# Autodesk Inventor assembly: Pancake_Top Board Assy
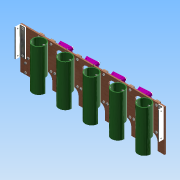
[picture p0: Inventor's stored thumbnail of the model, 180x180]
Saved by Autodesk Inventor 2018.1 (Build 221171000, 171)
## iProperties
Created: 2019-02-21
Part Number: Pancake_Top Board Assy
Document SubType Name: Assembly
Designer: James
Author: James
## Documents named in this file (18)
- C:\Users\admin\Desktop\Ball-Machine\Pancake Sort\Pancake_Top Board Assy.iam
- C:\Users\admin\Desktop\Ball-Machine\Pancake Sort\Pancake_Top Board.ipt
- C:\Users\admin\Desktop\Ball-Machine\Pancake Sort\Pancake_Angle Bracket 2.ipt
- C:\Users\admin\Desktop\Ball-Machine\Pancake Sort\Nyloc Nut - M4.ipt
- C:\Users\admin\Desktop\Ball-Machine\Pancake Sort\Socket Csk Screw - (A2) - M4 x  12.ipt
- C:\Users\admin\Desktop\Ball-Machine\Pancake Sort\Pancake_Side Piece.ipt
- C:\Users\admin\Desktop\Ball-Machine\Pancake Sort\Socket Csk Screw - (A2) - M4 x  16.ipt
- C:\Users\admin\Desktop\Ball-Machine\Pancake Sort\Pancake_Side Piece Short.ipt
- C:\Users\admin\Desktop\Ball-Machine\Pancake Sort\Pancake_Lower Pipe.ipt
- C:\Users\admin\Desktop\Ball-Machine\Pancake Sort\Pancake_Side Piece Short 2.ipt
- C:\Users\admin\Desktop\Ball-Machine\Pancake Sort\Socket Csk Screw - (A2) - M4 x  20.ipt
- C:\Users\admin\Desktop\Ball-Machine\Pancake Sort\Pancake_Side Piece Short 3.ipt
- C:\Users\admin\Desktop\Ball-Machine\Pancake Sort\Pancake_Switch Lever.ipt
- C:\Users\admin\Desktop\Ball-Machine\Pancake Sort\Pancake_Lever Mount Piece.ipt
- C:\Users\admin\Desktop\Ball-Machine\Selection Sort\Selection_Washer.ipt
- C:\Users\admin\Desktop\Ball-Machine\Pancake Sort\Socket Csk Screw - (A2) - M3 x  10.ipt
- C:\Users\admin\Desktop\Ball-Machine\Pancake Sort\Socket Cap Screw - Standard - (A2) - M3 x 8.ipt
- C:\Users\admin\Desktop\Ball-Machine\Pancake Sort\Pancake_Eye Screw.ipt
## Components (126 placed, 17 different names)
1. Pancake_Top Board:1 — Flush:1, Flush:2, Flush:3, Mate:1, Mate:2, Mate:3, Flush:4, Mate:4, Mate:5, Mate:6, Flush:5, Mate:7, Mate:8, Tangent:1, Tangent:2, Mate:13, Mate:14, Tangent:3, Tangent:4, Mate:19, Mate:20, Mate:21, Flush:6, Mate:24, Mate:25, Mate:28, Mate:29, Mate:30, Mate:35, Mate:36, Tangent:9, Mate:37, Mate:38, Angle:1, Mate:41, Mate:42, Tangent:10, Tangent:11, Mate:43, Mate:44, Mate:45, Mate:46, Mate:47, Mate:48, Mate:49, Mate:50, Mate:53, Mate:54, Mate:55, Mate:60, Mate:61, Mate:63, Mate:76, Mate:77, Mate:81, Tangent:19, Mate:84, Mate:85, Mate:86, Mate:87
2. Pancake_Angle Bracket 2:1 — Mate:1, Mate:2, Mate:3, Flush:4, Mate:9, Mate:10
3. Pancake_Angle Bracket 2:2 — Mate:4, Mate:5, Mate:6, Flush:5, Mate:15, Mate:16
4. Pancake_Side Piece Short 2:1 — Mate:44, Mate:45, Mate:46, Tangent:12, Tangent:13
5. Nyloc Nut - M4:35 — Mate:49, Mate:52
6. Socket Csk Screw - (A2) - M4 x  16:11 — Mate:47, Tangent:12, Mate:51
7. Nyloc Nut - M4:36 — Mate:50, Mate:51
8. Socket Csk Screw - (A2) - M4 x  16:12 — Mate:48, Tangent:13, Mate:52
9. Pancake_Side Piece Short 3:1 — Mate:53, Mate:54, Mate:55, Mate:58, Mate:59, Tangent:14, Tangent:15
10. Socket Csk Screw - (A2) - M4 x  16:13 — Mate:58, Tangent:14
11. Nyloc Nut - M4:37 — Mate:61
12. Socket Csk Screw - (A2) - M4 x  16:14 — Mate:59, Tangent:15
13. Nyloc Nut - M4:38 — Mate:60
14. Nyloc Nut - M4:1 — Mate:9, Mate:12
15. Nyloc Nut - M4:2 — Mate:10, Mate:11
16. Nyloc Nut - M4:3 — Mate:16, Mate:18
17. Nyloc Nut - M4:4 — Mate:15, Mate:17
18. Socket Csk Screw - (A2) - M4 x  12:1 — Mate:7, Tangent:1, Mate:11
19. Socket Csk Screw - (A2) - M4 x  12:2 — Mate:8, Tangent:2, Mate:12
20. Socket Csk Screw - (A2) - M4 x  12:3 — Mate:14, Tangent:3, Mate:17
21. Socket Csk Screw - (A2) - M4 x  12:4 — Mate:13, Tangent:4, Mate:18
22. Socket Csk Screw - (A2) - M4 x  16:2 — Mate:23, Tangent:5, Mate:27
23. Nyloc Nut - M4:6 — Mate:25, Mate:27
24. Socket Csk Screw - (A2) - M4 x  16:1 — Mate:22, Tangent:6, Mate:26
25. Nyloc Nut - M4:5 — Mate:24, Mate:26
26. Pancake_Side Piece:1 — Mate:19, Mate:20, Mate:21, Flush:6, Mate:22, Mate:23, Tangent:5, Tangent:6
27. Socket Csk Screw - (A2) - M4 x  16:3
28. Nyloc Nut - M4:7
29. Socket Csk Screw - (A2) - M4 x  16:4
30. Nyloc Nut - M4:8
31. Pancake_Side Piece:2 — Tangent:16
32. Socket Csk Screw - (A2) - M4 x  16:5
33. Nyloc Nut - M4:9
34. Socket Csk Screw - (A2) - M4 x  16:6
35. Nyloc Nut - M4:10
36. Pancake_Side Piece:3
37. Socket Csk Screw - (A2) - M4 x  16:7
38. Nyloc Nut - M4:11
39. Socket Csk Screw - (A2) - M4 x  16:8
40. Nyloc Nut - M4:12
41. Pancake_Side Piece:4
42. Socket Csk Screw - (A2) - M4 x  16:9
43. Nyloc Nut - M4:13
44. Socket Csk Screw - (A2) - M4 x  16:10
45. Nyloc Nut - M4:14
46. Pancake_Side Piece:5
47. Pancake_Side Piece Short:1 — Mate:28, Mate:29, Mate:30, Mate:33, Mate:34, Tangent:7, Tangent:8
48. Nyloc Nut - M4:15 — Mate:36
49. Socket Csk Screw - (A2) - M4 x  20:1 — Mate:34, Tangent:7
50. Nyloc Nut - M4:16 — Mate:35
51. Socket Csk Screw - (A2) - M4 x  20:6 — Mate:33, Tangent:8
52. Pancake_Side Piece Short:2 — Tangent:18, Mate:88, Mate:89
53. Nyloc Nut - M4:17
54. Socket Csk Screw - (A2) - M4 x  20:2
55. Nyloc Nut - M4:18
56. Socket Csk Screw - (A2) - M4 x  20:7
57. Pancake_Side Piece Short:3
58. Nyloc Nut - M4:19
59. Socket Csk Screw - (A2) - M4 x  20:3
60. Nyloc Nut - M4:20
61. Socket Csk Screw - (A2) - M4 x  20:8
62. Pancake_Side Piece Short:4
63. Nyloc Nut - M4:21
64. Socket Csk Screw - (A2) - M4 x  20:4
65. Nyloc Nut - M4:22
66. Socket Csk Screw - (A2) - M4 x  20:9
67. Pancake_Side Piece Short:5
68. Nyloc Nut - M4:23
69. Socket Csk Screw - (A2) - M4 x  20:5
70. Nyloc Nut - M4:24
71. Socket Csk Screw - (A2) - M4 x  20:10
72. Socket Csk Screw - (A2) - M4 x  12:6 — Mate:42, Tangent:11
73. Nyloc Nut - M4:26 — Mate:43, Flush:8
74. Socket Csk Screw - (A2) - M4 x  12:5 — Mate:41, Tangent:10
75. Nyloc Nut - M4:25 — Flush:8
76. Pancake_Lower Pipe:1 — Tangent:9, Mate:37, Mate:38, Angle:1
77. Socket Csk Screw - (A2) - M4 x  12:7
78. Nyloc Nut - M4:27
79. Socket Csk Screw - (A2) - M4 x  12:8
80. Nyloc Nut - M4:28
81. Pancake_Lower Pipe:2
82. Socket Csk Screw - (A2) - M4 x  12:9
83. Nyloc Nut - M4:29
84. Socket Csk Screw - (A2) - M4 x  12:10
85. Nyloc Nut - M4:30
86. Pancake_Lower Pipe:3
87. Socket Csk Screw - (A2) - M4 x  12:11
88. Nyloc Nut - M4:31
89. Socket Csk Screw - (A2) - M4 x  12:12
90. Nyloc Nut - M4:32
91. Pancake_Lower Pipe:4
92. Socket Csk Screw - (A2) - M4 x  12:13
93. Nyloc Nut - M4:33
94. Socket Csk Screw - (A2) - M4 x  12:14
95. Nyloc Nut - M4:34
96. Pancake_Lower Pipe:5
97. Socket Cap Screw - Standard - (A2) - M3 x 8:1 — Mate:82, Mate:83
98. Selection_Washer:2 — Mate:78, Mate:79, Mate:82, Mate:83
99. Pancake_Switch Lever:1 — Mate:63, Tangent:16, Tangent:18, Mate:80
100. Socket Csk Screw - (A2) - M3 x  10:2 — Mate:81, Tangent:19
101. Pancake_Lever Mount Piece:2 — Mate:76, Mate:77, Mate:78, Mate:79, Mate:80
102. Pancake_Eye Screw:7 — Mate:88, Mate:89
103. Socket Cap Screw - Standard - (A2) - M3 x 8:2
104. Selection_Washer:3
105. Pancake_Switch Lever:2
106. Socket Csk Screw - (A2) - M3 x  10:3
107. Pancake_Lever Mount Piece:3
108. Pancake_Eye Screw:8
109. Socket Cap Screw - Standard - (A2) - M3 x 8:3
110. Selection_Washer:4
111. Pancake_Switch Lever:3
112. Socket Csk Screw - (A2) - M3 x  10:4
113. Pancake_Lever Mount Piece:4
114. Pancake_Eye Screw:9
115. Socket Cap Screw - Standard - (A2) - M3 x 8:4
116. Selection_Washer:5
117. Pancake_Switch Lever:4
118. Socket Csk Screw - (A2) - M3 x  10:5
119. Pancake_Lever Mount Piece:5
120. Pancake_Eye Screw:10
121. Pancake_Eye Screw:1 — Mate:84, Mate:85
122. Pancake_Eye Screw:2 — Mate:86, Mate:87
123. Pancake_Eye Screw:3
124. Pancake_Eye Screw:4
125. Pancake_Eye Screw:5
126. Pancake_Eye Screw:6
## Component patterns: (5 elements, first: Socket Csk Screw - (A2) - M4 x  16:2 + Nyloc Nut - M4:6 + Socket Csk Screw - (A2) - M4 x  16:1 + Nyloc Nut - M4:5 + Pancake_Side Piece:1), (5 elements, first: Pancake_Side Piece Short:1 + Nyloc Nut - M4:15 + Socket Csk Screw - (A2) - M4 x  20:1 + Nyloc Nut - M4:16 + Socket Csk Screw - (A2) - M4 x  20:6), (5 elements, first: Socket Csk Screw - (A2) - M4 x  12:6 + Nyloc Nut - M4:26 + Socket Csk Screw - (A2) - M4 x  12:5 + Nyloc Nut - M4:25 + Pancake_Lower Pipe:1), (4 elements, first: Socket Cap Screw - Standard - (A2) - M3 x 8:1 + Selection_Washer:2 + Pancake_Switch Lever:1 + Socket Csk Screw - (A2) - M3 x  10:2 + Pancake_Lever Mount Piece:2 + Pancake_Eye Screw:7), (3 elements, first: Pancake_Eye Screw:1 + Pancake_Eye Screw:2)
## Relationships (102: Mate 76, Tangent 18, Flush 7, Angle 1)
- Flush:1: Pancake_Top Board:1
- Flush:2: Pancake_Top Board:1
- Flush:3: Pancake_Top Board:1
- Mate:1: Pancake_Top Board:1 ↔ Pancake_Angle Bracket 2:1
- Mate:2: Pancake_Top Board:1 ↔ Pancake_Angle Bracket 2:1
- Mate:3: Pancake_Top Board:1 ↔ Pancake_Angle Bracket 2:1
- Flush:4: Pancake_Top Board:1 ↔ Pancake_Angle Bracket 2:1
- Mate:4: Pancake_Top Board:1 ↔ Pancake_Angle Bracket 2:2
- Mate:5: Pancake_Top Board:1 ↔ Pancake_Angle Bracket 2:2
- Mate:6: Pancake_Top Board:1 ↔ Pancake_Angle Bracket 2:2
- Flush:5: Pancake_Top Board:1 ↔ Pancake_Angle Bracket 2:2
- Mate:7: Pancake_Top Board:1 ↔ Socket Csk Screw - (A2) - M4 x  12:1
- Mate:8: Pancake_Top Board:1 ↔ Socket Csk Screw - (A2) - M4 x  12:2
- Tangent:1: Pancake_Top Board:1 ↔ Socket Csk Screw - (A2) - M4 x  12:1
- Tangent:2: Pancake_Top Board:1 ↔ Socket Csk Screw - (A2) - M4 x  12:2
- Mate:9: Pancake_Angle Bracket 2:1 ↔ Nyloc Nut - M4:1
- Mate:10: Pancake_Angle Bracket 2:1 ↔ Nyloc Nut - M4:2
- Mate:11: Nyloc Nut - M4:2 ↔ Socket Csk Screw - (A2) - M4 x  12:1
- Mate:12: Nyloc Nut - M4:1 ↔ Socket Csk Screw - (A2) - M4 x  12:2
- Mate:13: Pancake_Top Board:1 ↔ Socket Csk Screw - (A2) - M4 x  12:4
- Mate:14: Pancake_Top Board:1 ↔ Socket Csk Screw - (A2) - M4 x  12:3
- Tangent:3: Pancake_Top Board:1 ↔ Socket Csk Screw - (A2) - M4 x  12:3
- Tangent:4: Pancake_Top Board:1 ↔ Socket Csk Screw - (A2) - M4 x  12:4
- Mate:15: Pancake_Angle Bracket 2:2 ↔ Nyloc Nut - M4:4
- Mate:16: Pancake_Angle Bracket 2:2 ↔ Nyloc Nut - M4:3
- Mate:17: Nyloc Nut - M4:4 ↔ Socket Csk Screw - (A2) - M4 x  12:3
- Mate:18: Nyloc Nut - M4:3 ↔ Socket Csk Screw - (A2) - M4 x  12:4
- Mate:19: Pancake_Top Board:1 ↔ Pancake_Side Piece:1
- Mate:20: Pancake_Top Board:1 ↔ Pancake_Side Piece:1
- Mate:21: Pancake_Top Board:1 ↔ Pancake_Side Piece:1
- Flush:6: Pancake_Top Board:1 ↔ Pancake_Side Piece:1
- Mate:22: Socket Csk Screw - (A2) - M4 x  16:1 ↔ Pancake_Side Piece:1
- Mate:23: Socket Csk Screw - (A2) - M4 x  16:2 ↔ Pancake_Side Piece:1
- Tangent:5: Socket Csk Screw - (A2) - M4 x  16:2 ↔ Pancake_Side Piece:1
- Tangent:6: Socket Csk Screw - (A2) - M4 x  16:1 ↔ Pancake_Side Piece:1
- Mate:24: Pancake_Top Board:1 ↔ Nyloc Nut - M4:5
- Mate:25: Pancake_Top Board:1 ↔ Nyloc Nut - M4:6
- Mate:26: Socket Csk Screw - (A2) - M4 x  16:1 ↔ Nyloc Nut - M4:5
- Mate:27: Socket Csk Screw - (A2) - M4 x  16:2 ↔ Nyloc Nut - M4:6
- Mate:28: Pancake_Top Board:1 ↔ Pancake_Side Piece Short:1
- Mate:29: Pancake_Top Board:1 ↔ Pancake_Side Piece Short:1
- Mate:30: Pancake_Top Board:1 ↔ Pancake_Side Piece Short:1
- [Mate]: Nyloc Nut - M4:15 ↔ Socket Csk Screw - (A2) - M4 x  20:1
- [Mate]: Nyloc Nut - M4:16 ↔ Socket Csk Screw - (A2) - M4 x  20:6
- Mate:33: Pancake_Side Piece Short:1 ↔ Socket Csk Screw - (A2) - M4 x  20:6
- Mate:34: Pancake_Side Piece Short:1 ↔ Socket Csk Screw - (A2) - M4 x  20:1
- Tangent:7: Pancake_Side Piece Short:1 ↔ Socket Csk Screw - (A2) - M4 x  20:1
- Tangent:8: Pancake_Side Piece Short:1 ↔ Socket Csk Screw - (A2) - M4 x  20:6
- Mate:35: Pancake_Top Board:1 ↔ Nyloc Nut - M4:16
- Mate:36: Pancake_Top Board:1 ↔ Nyloc Nut - M4:15
- Tangent:9: Pancake_Top Board:1 ↔ Pancake_Lower Pipe:1
- Mate:37: Pancake_Top Board:1 ↔ Pancake_Lower Pipe:1
- Mate:38: Pancake_Top Board:1 ↔ Pancake_Lower Pipe:1
- Angle:1 (180 deg): Pancake_Top Board:1 ↔ Pancake_Lower Pipe:1
- [Mate]: Socket Csk Screw - (A2) - M4 x  12:5 ↔ Nyloc Nut - M4:25
- [Mate]: Socket Csk Screw - (A2) - M4 x  12:6 ↔ Nyloc Nut - M4:26
- Mate:41: Pancake_Top Board:1 ↔ Socket Csk Screw - (A2) - M4 x  12:5
- Mate:42: Pancake_Top Board:1 ↔ Socket Csk Screw - (A2) - M4 x  12:6
- Tangent:10: Pancake_Top Board:1 ↔ Socket Csk Screw - (A2) - M4 x  12:5
- Tangent:11: Pancake_Top Board:1 ↔ Socket Csk Screw - (A2) - M4 x  12:6
- Mate:43 (3 mm): Pancake_Top Board:1 ↔ Nyloc Nut - M4:26
- Flush:8: Nyloc Nut - M4:26 ↔ Nyloc Nut - M4:25
- Mate:44: Pancake_Top Board:1 ↔ Pancake_Side Piece Short 2:1
- Mate:45: Pancake_Top Board:1 ↔ Pancake_Side Piece Short 2:1
- Mate:46: Pancake_Top Board:1 ↔ Pancake_Side Piece Short 2:1
- Mate:47: Pancake_Top Board:1 ↔ Socket Csk Screw - (A2) - M4 x  16:11
- Mate:48: Pancake_Top Board:1 ↔ Socket Csk Screw - (A2) - M4 x  16:12
- Tangent:12: Pancake_Side Piece Short 2:1 ↔ Socket Csk Screw - (A2) - M4 x  16:11
- Tangent:13: Pancake_Side Piece Short 2:1 ↔ Socket Csk Screw - (A2) - M4 x  16:12
- Mate:49: Pancake_Top Board:1 ↔ Nyloc Nut - M4:35
- Mate:50: Pancake_Top Board:1 ↔ Nyloc Nut - M4:36
- Mate:51: Socket Csk Screw - (A2) - M4 x  16:11 ↔ Nyloc Nut - M4:36
- Mate:52: Nyloc Nut - M4:35 ↔ Socket Csk Screw - (A2) - M4 x  16:12
- Mate:53: Pancake_Top Board:1 ↔ Pancake_Side Piece Short 3:1
- Mate:54: Pancake_Top Board:1 ↔ Pancake_Side Piece Short 3:1
- Mate:55: Pancake_Top Board:1 ↔ Pancake_Side Piece Short 3:1
- [Mate]: Socket Csk Screw - (A2) - M4 x  16:13 ↔ Nyloc Nut - M4:37
- [Mate]: Socket Csk Screw - (A2) - M4 x  16:14 ↔ Nyloc Nut - M4:38
- Mate:58: Pancake_Side Piece Short 3:1 ↔ Socket Csk Screw - (A2) - M4 x  16:13
- Mate:59: Pancake_Side Piece Short 3:1 ↔ Socket Csk Screw - (A2) - M4 x  16:14
- Tangent:14: Pancake_Side Piece Short 3:1 ↔ Socket Csk Screw - (A2) - M4 x  16:13
- Tangent:15: Pancake_Side Piece Short 3:1 ↔ Socket Csk Screw - (A2) - M4 x  16:14
- Mate:60: Pancake_Top Board:1 ↔ Nyloc Nut - M4:38
- Mate:61: Pancake_Top Board:1 ↔ Nyloc Nut - M4:37
- Mate:63: Pancake_Top Board:1 ↔ Pancake_Switch Lever:1
- Tangent:16: Pancake_Side Piece:2 ↔ Pancake_Switch Lever:1
- Tangent:18: Pancake_Side Piece Short:2 ↔ Pancake_Switch Lever:1
- Mate:76: Pancake_Top Board:1 ↔ Pancake_Lever Mount Piece:2
- Mate:77: Pancake_Top Board:1 ↔ Pancake_Lever Mount Piece:2
- Mate:78: Selection_Washer:2 ↔ Pancake_Lever Mount Piece:2
- Mate:79: Selection_Washer:2 ↔ Pancake_Lever Mount Piece:2
- Mate:80: Pancake_Switch Lever:1 ↔ Pancake_Lever Mount Piece:2
- Mate:81: Pancake_Top Board:1 ↔ Socket Csk Screw - (A2) - M3 x  10:2
- Tangent:19: Pancake_Top Board:1 ↔ Socket Csk Screw - (A2) - M3 x  10:2
- Mate:82: Socket Cap Screw - Standard - (A2) - M3 x 8:1 ↔ Selection_Washer:2
- Mate:83: Socket Cap Screw - Standard - (A2) - M3 x 8:1 ↔ Selection_Washer:2
- Mate:84: Pancake_Top Board:1 ↔ Pancake_Eye Screw:1
- Mate:85: Pancake_Top Board:1 ↔ Pancake_Eye Screw:1
- Mate:86: Pancake_Top Board:1 ↔ Pancake_Eye Screw:2
- Mate:87: Pancake_Top Board:1 ↔ Pancake_Eye Screw:2
- Mate:88: Pancake_Side Piece Short:2 ↔ Pancake_Eye Screw:7
- Mate:89: Pancake_Side Piece Short:2 ↔ Pancake_Eye Screw:7
## Named parameters: d47_d39 = 0 mm, d48_d39 = 0 mm, d63_d18 = 0 mm, d64_d18 = 0 mm, d89_d84 = 0 mm, d90_d84 = 0 mm
